# Autodesk Inventor assembly: EnsamblajeBase
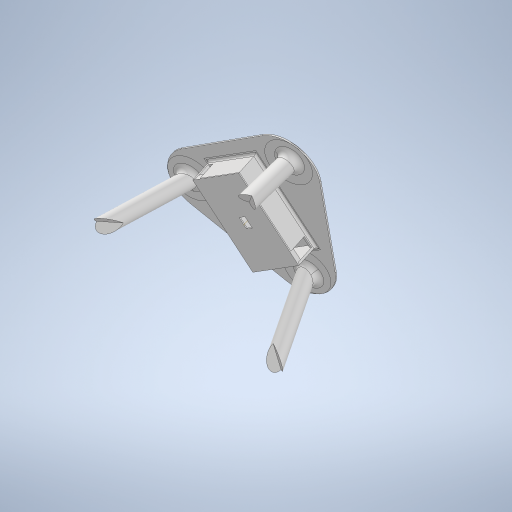
[picture p0: Inventor's stored thumbnail of the model, 512x512]
Saved by Autodesk Inventor 2024 (Build 280153000, 153)
## iProperties
Created: 2024-07-14
Part Number: EnsamblajeBase
Document SubType Name: Assembly
Designer: sergi
Author: sergi
## Documents named in this file (6)
- C:\Users\sergi\OneDrive\Escritorio\proyectos\Piso\Dodecaedro\EnsamblajeBase.iam
- C:\Users\sergi\OneDrive\Documentos\Base4.ipt
- C:\Users\sergi\OneDrive\Escritorio\proyectos\Piso\Dodecaedro\Base4Baterias.ipt
- C:\Users\sergi\OneDrive\Escritorio\proyectos\Piso\Dodecaedro\TapaBaterias.ipt
- C:\Users\sergi\OneDrive\Escritorio\proyectos\Piso\Dodecaedro\Dodecaedro.ipt
- C:\Users\sergi\OneDrive\Escritorio\proyectos\Piso\Dodecaedro\Brazos.ipt
## Components (5 placed, 5 different names)
1. Base4:1 — Coincidencia:12, Coincidencia:16, Coincidencia:17, Coincidencia:18, Coincidencia:20, Coincidencia:23, Nivelación:4
2. Base4Baterias:1 — Coincidencia:17, Coincidencia:18, Nivelación:2, Nivelación:3, Coincidencia:19
3. TapaBaterias:1 — Nivelación:2, Nivelación:3, Coincidencia:19
4. Dodecaedro:1 — Coincidencia:12, Coincidencia:20, Coincidencia:23, Nivelación:5, Nivelación:6, Nivelación:7
5. Brazos:1 — Nivelación:4, Nivelación:5, Nivelación:6, Nivelación:7
## Relationships (13: Mate 7, Flush 6)
- Coincidencia:12 [Mate]: Base4:1 ↔ Dodecaedro:1
- Coincidencia:16 [Mate] (72.1 mm): Base4:1
- Coincidencia:17 [Mate]: Base4:1 ↔ Base4Baterias:1
- Coincidencia:18 [Mate]: Base4:1 ↔ Base4Baterias:1
- Nivelación:2 [Flush]: Base4Baterias:1 ↔ TapaBaterias:1
- Nivelación:3 [Flush]: Base4Baterias:1 ↔ TapaBaterias:1
- Coincidencia:19 [Mate]: Base4Baterias:1 ↔ TapaBaterias:1
- Coincidencia:20 [Mate] (72.1 mm): Base4:1 ↔ Dodecaedro:1
- Coincidencia:23 [Mate]: Base4:1 ↔ Dodecaedro:1
- Nivelación:4 [Flush]: Base4:1 ↔ Brazos:1
- Nivelación:5 [Flush]: Dodecaedro:1 ↔ Brazos:1
- Nivelación:6 [Flush]: Dodecaedro:1 ↔ Brazos:1
- Nivelación:7 [Flush]: Dodecaedro:1 ↔ Brazos:1
